# Autodesk Inventor assembly: ShooterAssemblyForRobotWithCamControl
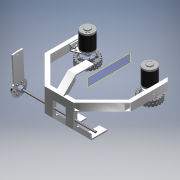
[picture p0: Inventor's stored thumbnail of the model, 180x180]
Saved by Autodesk Inventor 2017 (Build 210142000, 142)
## iProperties
Created: 2016-02-07
Part Number: ShooterAssemblyForRobotWithCamControl
Document SubType Name: Assembly
Designer: steele
Author: steele
## Documents named in this file (10)
- C:\snobotics\CAD-Development\robSteele\SnoBotics2016\2016-05-05-ShooterPrototype\ShooterAssemblyForRobotWithCamControl.iam
- C:\snobotics\CAD-Development\robSteele\SnoBotics2016\2016-05-05-ShooterPrototype\Mini_CIM_MotorHub_4_inch_wheel.iam
- C:\snobotics\CAD-Development\robSteele\SnoBotics2016\2016-05-05-ShooterPrototype\CIM_MotorHub_4_inch_wheel.iam
- C:\snobotics\CAD-Development\robSteele\SnoBotics2016\2016-05-05-ShooterPrototype\ShooterFrameAssembly05.iam
- C:\snobotics\CAD-Development\robSteele\SnoBotics2016\AM Parts\am-0134a+375+Key+Hub+r2.ipt
- C:\snobotics\CAD-Development\robSteele\SnoBotics2016\2016-05-05-ShooterPrototype\ShooterAssemblyForRobotV16\Design Accelerator\Bolted Connection1.iam
- C:\snobotics\CAD-Development\robSteele\SnoBotics2016\2016-05-05-ShooterPrototype\ShooterAssemblyForRobotV16\Design Accelerator\Bolted Connection2.iam
- C:\snobotics\CAD-Development\robSteele\SnoBotics2016\2016-05-05-ShooterPrototype\SteelRodForShooter.ipt
- C:\snobotics\CAD-Development\robSteele\SnoBotics2016\2016-05-05-ShooterPrototype\camPlate.ipt
- C:\snobotics\CAD-Development\robSteele\SnoBotics2016\2016-05-05-ShooterPrototype\ShooterAssemblyForRobotWithCamControl\Design Accelerator\Bolted Connection1.iam
## Components (14 placed, 7 different names)
1. ShooterFrameAssembly05:1 [sub-assembly] — Mate:1, Mate:16, Flush:6, Mate:17, Insert:4, Mate:18, Mate:19
2. Mini_CIM_MotorHub_4_inch_wheel:1 [sub-assembly] — Mate:1, Flush:5, Mate:16, Flush:6, Flush:7, Flush:8, Mate:20, Mate:21
3. SteelRodForShooter:1 — Insert:4, Insert:5
4. CIM_MotorHub_4_inch_wheel:1 [sub-assembly] — Flush:5, Mate:17, Flush:7, Flush:8
5. am-0134a+375+Key+Hub+r2:1 — Insert:5, Insert:6
6. Bolted Connection:1 [sub-assembly] — Mate:18, Mate:19
7. Bolted Connection:2 [sub-assembly] — Mate:20, Mate:21
8. camPlate:1 — Insert:6, Mate:22, Mate:23
9. Bolted Connection:3 [sub-assembly] — Mate:22, Mate:23
10. Bolted Connection:4 [sub-assembly]
11. Bolted Connection:5 [sub-assembly]
12. Bolted Connection:6 [sub-assembly]
13. Bolted Connection:7 [sub-assembly]
14. Bolted Connection:8 [sub-assembly]
## Component patterns: (6 elements, first: Bolted Connection:3)
## Relationships (16: Mate 9, Flush 4, Insert 3)
- Mate:1: ShooterFrameAssembly05:1 ↔ Mini_CIM_MotorHub_4_inch_wheel:1
- Flush:5: Mini_CIM_MotorHub_4_inch_wheel:1 ↔ CIM_MotorHub_4_inch_wheel:1
- Mate:16: ShooterFrameAssembly05:1 ↔ Mini_CIM_MotorHub_4_inch_wheel:1
- Flush:6 (-4.7625 mm): ShooterFrameAssembly05:1 ↔ Mini_CIM_MotorHub_4_inch_wheel:1
- Mate:17: ShooterFrameAssembly05:1 ↔ CIM_MotorHub_4_inch_wheel:1
- Flush:7: Mini_CIM_MotorHub_4_inch_wheel:1 ↔ CIM_MotorHub_4_inch_wheel:1
- Flush:8: Mini_CIM_MotorHub_4_inch_wheel:1 ↔ CIM_MotorHub_4_inch_wheel:1
- Insert:4 (101.6 mm): ShooterFrameAssembly05:1 ↔ SteelRodForShooter:1
- Insert:5: SteelRodForShooter:1 ↔ am-0134a+375+Key+Hub+r2:1
- Mate:18: ShooterFrameAssembly05:1 ↔ Bolted Connection:1
- Mate:19: ShooterFrameAssembly05:1 ↔ Bolted Connection:1
- Mate:20: Mini_CIM_MotorHub_4_inch_wheel:1 ↔ Bolted Connection:2
- Mate:21: Mini_CIM_MotorHub_4_inch_wheel:1 ↔ Bolted Connection:2
- Insert:6: am-0134a+375+Key+Hub+r2:1 ↔ camPlate:1
- Mate:22: camPlate:1 ↔ Bolted Connection:3
- Mate:23: camPlate:1 ↔ Bolted Connection:3
